# Autodesk Inventor assembly: Remote Assembly
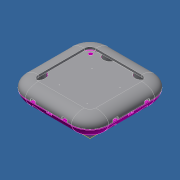
[picture p0: Inventor's stored thumbnail of the model, 180x180]
Saved by Autodesk Inventor 2016 (Build 200138000, 138)
## iProperties
Created: 2015-06-16
Part Number: Remote Assembly
Document SubType Name: Assembly
Designer: Samuel Clay
Author: Samuel Clay
## Documents named in this file (7)
- Z:\turntouch\remote\enclosure\inventor\Remote Assembly.iam
- Z:\turntouch\remote\enclosure\inventor\Remote Top.ipt
- Z:\turntouch\remote\enclosure\inventor\Remote Bottom.ipt
- Z:\turntouch\remote\enclosure\inventor\Remote Buttons.ipt
- Z:\turntouch\remote\enclosure\inventor\Remote Buttons Export.ipt
- Z:\turntouch\remote\enclosure\inventor\Eagle PCB.ipt
- Z:\turntouch\remote\enclosure\inventor\Eagle PCB rev 21.ipt
## Components (6 placed, 6 different names)
1. Remote Top:1 — Flush:1
2. Remote Bottom:1 — Mate:1, Rotational:1
3. Remote Buttons:1 — Flush:1
4. Remote Buttons Export:1
5. Eagle PCB:1 — Mate:1
6. Eagle PCB rev 21:1 — Rotational:1
## Relationships (3: Flush 1, Mate 1, RevoluteJoint 1)
- Flush:1: Remote Top:1 ↔ Remote Buttons:1
- Mate:1: Remote Bottom:1 ↔ Eagle PCB:1
- Rotational:1 [RevoluteJoint]: Remote Bottom:1 ↔ Eagle PCB rev 21:1
